# Autodesk Inventor assembly: WheelFeeder
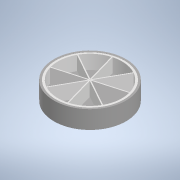
[picture p0: Inventor's stored thumbnail of the model, 180x180]
Saved by Autodesk Inventor 2020 (Build 240168000, 168)
## iProperties
Created: 2020-03-05
Part Number: WheelFeeder
Document SubType Name: Assembly
Designer: jared.jones280
Author: jared.jones280
## Documents named in this file (3)
- \\toaster\homes\j\a\jared.jones280\nt\Autodesk\WheelFeeder.iam
- \\toaster\homes\j\a\jared.jones280\nt\Autodesk\FeedWheelShell.ipt
- \\toaster\homes\j\a\jared.jones280\nt\Autodesk\FeedWheel.ipt
## Components (2 placed, 2 different names)
1. FeedWheelShell:1 — Mate:1, Flush:1
2. FeedWheel:1 — Mate:1, Flush:1
## Relationships (2: Mate 1, Flush 1)
- Mate:1: FeedWheelShell:1 ↔ FeedWheel:1
- Flush:1: FeedWheelShell:1 ↔ FeedWheel:1
